# Autodesk Inventor assembly: ServoHolder
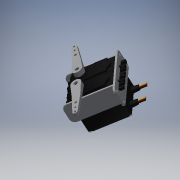
[picture p0: Inventor's stored thumbnail of the model, 180x180]
Saved by Autodesk Inventor 2018.2 (Build 222227000, 227)
## iProperties
Created: 2018-02-17
Part Number: ServoHolder
Material: Generisch
Document SubType Name: Assembly
Designer: JochenAlt
Author: JochenAlt
## Documents named in this file (4)
- D:\Projects\PrivateDancer\CAD\ServoHolder.iam
- D:\Projects\PrivateDancer\CAD\hitec-hs-645mg\HS-645 MG.ipt
- D:\Projects\PrivateDancer\CAD\Stewart-Holder.ipt
- D:\Projects\PrivateDancer\CAD\ServoArm 38mm.ipt
## Components (5 placed, 3 different names)
1. HS-645 MG:1 — Passend:3, Passend:9, Passend:12, Passend:14, Passend:17
2. HS-645 MG:2 — Passend:1, Passend:8, Passend:13, Passend:15, Passend:16
3. Stewart-Holder:1 — Passend:1, Passend:3, Passend:8, Passend:9, Passend:16, Passend:17
4. ServoArm:1 — Passend:12, Passend:14
5. ServoArm:2 — Passend:13, Passend:15
## Relationships (10: Mate 10)
- Passend:1 [Mate] (0.3 mm): HS-645 MG:2 ↔ Stewart-Holder:1
- Passend:3 [Mate] (0.3 mm): HS-645 MG:1 ↔ Stewart-Holder:1
- Passend:8 [Mate] (0.3 mm): HS-645 MG:2 ↔ Stewart-Holder:1
- Passend:9 [Mate] (0.3 mm): HS-645 MG:1 ↔ Stewart-Holder:1
- Passend:12 [Mate]: HS-645 MG:1 ↔ ServoArm:1
- Passend:13 [Mate]: HS-645 MG:2 ↔ ServoArm:2
- Passend:14 [Mate] (0.4 mm): HS-645 MG:1 ↔ ServoArm:1
- Passend:15 [Mate] (0.3 mm): HS-645 MG:2 ↔ ServoArm:2
- Passend:16 [Mate] (0.3 mm): HS-645 MG:2 ↔ Stewart-Holder:1
- Passend:17 [Mate] (0.3 mm): HS-645 MG:1 ↔ Stewart-Holder:1
